# Autodesk Inventor assembly: motor_bench_stand
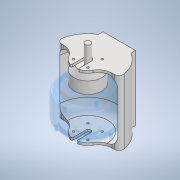
[picture p0: Inventor's stored thumbnail of the model, 180x180]
Saved by Autodesk Inventor 2022.6 (Build 266554010, 554A)
## iProperties
Created: 2025-03-25
Part Number: motor_bench_stand
Document SubType Name: Assembly
Designer: gakut
Author: gakut
## Documents named in this file (4)
- C:\Users\gakut\Documents\Inventor\gakutasu_default_cad\motor_bench_stand\motor_bench_stand.iam
- C:\Users\gakut\Documents\Inventor\gakutasu_default_cad\motor_bench_stand\movero.ipt
- C:\Users\gakut\Documents\Inventor\gakutasu_default_cad\motor_bench_stand\encoder_mount.ipt
- C:\Users\gakut\Documents\Inventor\gakutasu_default_cad\motor_bench_stand\encoder_shaft.ipt
## Components (3 placed, 3 different names)
1. movero:1 — メイト:1, メイト:2, メイト:3, メイト:4, メイト:5
2. encoder_mount:1 — メイト:1, メイト:2, メイト:5
3. encoder_shaft:1 — メイト:3, メイト:4
## Relationships (5: Mate 5)
- メイト:1 [Mate]: movero:1 ↔ encoder_mount:1
- メイト:2 [Mate]: movero:1 ↔ encoder_mount:1
- メイト:3 [Mate]: movero:1 ↔ encoder_shaft:1
- メイト:4 [Mate]: movero:1 ↔ encoder_shaft:1
- メイト:5 [Mate]: movero:1 ↔ encoder_mount:1
